# Autodesk Inventor assembly: door
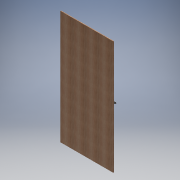
[picture p0: Inventor's stored thumbnail of the model, 180x180]
Saved by Autodesk Inventor 2019 (Build 230136000, 136)
## iProperties
Created: 2018-07-30
Part Number: door
Document SubType Name: Assembly
Designer: User
Author: User
## Documents named in this file (3)
- C:\Users\User\Documents\GitHub\darkRadio\3D Models\Room Model\door.iam
- C:\Users\User\Documents\GitHub\darkRadio\3D Models\Room Model\door_base.ipt
- C:\Users\User\Documents\GitHub\darkRadio\3D Models\Room Model\door_handle.ipt
## Components (2 placed, 2 different names)
1. door_base:1 — Mate:1, Flush:1, Flush:2
2. door_handle:1 — Mate:1, Flush:1, Flush:2
## Relationships (3: Flush 2, Mate 1)
- Mate:1: door_base:1 ↔ door_handle:1
- Flush:1: door_base:1 ↔ door_handle:1
- Flush:2 (183.9 mm): door_base:1 ↔ door_handle:1
